# Autodesk Inventor assembly: ThermaShield
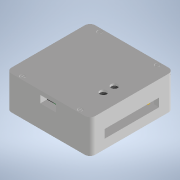
[picture p0: Inventor's stored thumbnail of the model, 180x180]
Saved by Autodesk Inventor 2022 (Build 260153000, 153)
## iProperties
Created: 2024-06-23
Part Number: ThermaShield
Document SubType Name: Assembly
Designer: Timur
Author: Timur
## Documents named in this file (8)
- B:\YandexDisk\YandexDisk\Учеба\НИУ ВШЭ\2 модуль\Проектный семинар\Финальный проект\Case\ThermaShield.iam
- B:\YandexDisk\YandexDisk\Учеба\НИУ ВШЭ\2 модуль\Проектный семинар\Финальный проект\Case\Case_Base.ipt
- B:\YandexDisk\YandexDisk\Учеба\НИУ ВШЭ\2 модуль\Проектный семинар\Финальный проект\Case\Threaded Insert - M2x4x3.5_Inventor.ipt
- B:\YandexDisk\YandexDisk\Учеба\НИУ ВШЭ\2 модуль\Проектный семинар\Финальный проект\Case\Стойка (M2x4)x5mm.ipt
- B:\YandexDisk\YandexDisk\Учеба\НИУ ВШЭ\2 модуль\Проектный семинар\Финальный проект\Case\Case_Cover.ipt
- B:\YandexDisk\YandexDisk\Учеба\НИУ ВШЭ\2 модуль\Проектный семинар\Финальный проект\Case\Винт M2-6gx6 ГОСТ 17475-80.ipt
- B:\YandexDisk\YandexDisk\Учеба\НИУ ВШЭ\2 модуль\Проектный семинар\Финальный проект\Case\Винт M2-6gx5 ГОСТ 1491-80.ipt
- B:\YandexDisk\YandexDisk\Учеба\НИУ ВШЭ\2 модуль\Проектный семинар\Финальный проект\Case\ThermaShield_V0.9\ThermaShield_V0.9.iam
## Components (23 placed, 7 different names)
1. Case_Base:1 — Совмещение:1, Заподлицо:1, Совмещение:2, Заподлицо:2, Совмещение:3, Заподлицо:3, Совмещение:4, Заподлицо:4, Совмещение:5, Совмещение:6, Совмещение:7, Совмещение:8, Заподлицо:5, Заподлицо:6, Заподлицо:7, Заподлицо:8, Заподлицо:9, Совмещение:20
2. Threaded Insert - M2x4x3.5_Inventor:1 — Совмещение:7, Заподлицо:7, Совмещение:12, Совмещение:13
3. Threaded Insert - M2x4x3.5_Inventor:2 — Совмещение:3, Заподлицо:3, Совмещение:22
4. Threaded Insert - M2x4x3.5_Inventor:3 — Совмещение:4, Заподлицо:4
5. Threaded Insert - M2x4x3.5_Inventor:4 — Совмещение:6, Заподлицо:6, Совмещение:11, Совмещение:14
6. Threaded Insert - M2x4x3.5_Inventor:5 — Совмещение:8, Заподлицо:8, Совмещение:10, Совмещение:15
7. Threaded Insert - M2x4x3.5_Inventor:6 — Совмещение:2, Заподлицо:2
8. Threaded Insert - M2x4x3.5_Inventor:7 — Совмещение:1, Заподлицо:1, Заподлицо:9, Совмещение:21
9. Threaded Insert - M2x4x3.5_Inventor:8 — Совмещение:5, Заподлицо:5, Совмещение:9, Совмещение:16
10. Стойка (M2x4)x5mm:1 — Совмещение:10, Совмещение:15
11. Стойка (M2x4)x5mm:2 — Совмещение:12, Совмещение:13, Совмещение:23, Совмещение:25
12. Стойка (M2x4)x5mm:3 — Совмещение:11, Совмещение:14
13. Стойка (M2x4)x5mm:4 — Совмещение:9, Совмещение:16
14. Case_Cover:1 — Совмещение:20, Совмещение:21, Совмещение:22, С поворотом:1, С поворотом:2, С поворотом:3, С поворотом:4
15. Винт ГОСТ 17475-80 M2 x 6:1 — С поворотом:4
16. Винт ГОСТ 17475-80 M2 x 6:2 — С поворотом:3
17. Винт ГОСТ 17475-80 M2 x 6:3 — С поворотом:2
18. Винт ГОСТ 17475-80 M2 x 6:4 — С поворотом:1
19. ThermaShield_V0.9:1 [sub-assembly] — Совмещение:23, Совмещение:25, Жесткий:1, Жесткий:2, С поворотом:5, Жесткий:3
20. Винт ГОСТ 1491-80 M 2 x 5:1 — С поворотом:5
21. Винт ГОСТ 1491-80 M 2 x 5:2 — Жесткий:1
22. Винт ГОСТ 1491-80 M 2 x 5:3 — Жесткий:3
23. Винт ГОСТ 1491-80 M 2 x 5:4 — Жесткий:2
## Relationships (38: Mate 21, Flush 9, RevoluteJoint 5, WeldJoint 3)
- Совмещение:1 [Mate]: Case_Base:1 ↔ Threaded Insert - M2x4x3.5_Inventor:7
- Заподлицо:1 [Flush]: Case_Base:1 ↔ Threaded Insert - M2x4x3.5_Inventor:7
- Совмещение:2 [Mate]: Case_Base:1 ↔ Threaded Insert - M2x4x3.5_Inventor:6
- Заподлицо:2 [Flush]: Case_Base:1 ↔ Threaded Insert - M2x4x3.5_Inventor:6
- Совмещение:3 [Mate]: Case_Base:1 ↔ Threaded Insert - M2x4x3.5_Inventor:2
- Заподлицо:3 [Flush]: Case_Base:1 ↔ Threaded Insert - M2x4x3.5_Inventor:2
- Совмещение:4 [Mate]: Case_Base:1 ↔ Threaded Insert - M2x4x3.5_Inventor:3
- Заподлицо:4 [Flush]: Case_Base:1 ↔ Threaded Insert - M2x4x3.5_Inventor:3
- Совмещение:5 [Mate]: Case_Base:1 ↔ Threaded Insert - M2x4x3.5_Inventor:8
- Совмещение:6 [Mate]: Case_Base:1 ↔ Threaded Insert - M2x4x3.5_Inventor:4
- Совмещение:7 [Mate]: Case_Base:1 ↔ Threaded Insert - M2x4x3.5_Inventor:1
- Совмещение:8 [Mate]: Case_Base:1 ↔ Threaded Insert - M2x4x3.5_Inventor:5
- Заподлицо:5 [Flush]: Case_Base:1 ↔ Threaded Insert - M2x4x3.5_Inventor:8
- Заподлицо:6 [Flush]: Case_Base:1 ↔ Threaded Insert - M2x4x3.5_Inventor:4
- Заподлицо:7 [Flush]: Case_Base:1 ↔ Threaded Insert - M2x4x3.5_Inventor:1
- Заподлицо:8 [Flush]: Case_Base:1 ↔ Threaded Insert - M2x4x3.5_Inventor:5
- Совмещение:9 [Mate]: Threaded Insert - M2x4x3.5_Inventor:8 ↔ Стойка (M2x4)x5mm:4
- Совмещение:10 [Mate]: Threaded Insert - M2x4x3.5_Inventor:5 ↔ Стойка (M2x4)x5mm:1
- Совмещение:11 [Mate]: Threaded Insert - M2x4x3.5_Inventor:4 ↔ Стойка (M2x4)x5mm:3
- Совмещение:12 [Mate]: Threaded Insert - M2x4x3.5_Inventor:1 ↔ Стойка (M2x4)x5mm:2
- Совмещение:13 [Mate]: Threaded Insert - M2x4x3.5_Inventor:1 ↔ Стойка (M2x4)x5mm:2
- Совмещение:14 [Mate]: Threaded Insert - M2x4x3.5_Inventor:4 ↔ Стойка (M2x4)x5mm:3
- Совмещение:15 [Mate]: Threaded Insert - M2x4x3.5_Inventor:5 ↔ Стойка (M2x4)x5mm:1
- Совмещение:16 [Mate]: Threaded Insert - M2x4x3.5_Inventor:8 ↔ Стойка (M2x4)x5mm:4
- Заподлицо:9 [Flush]: Case_Base:1 ↔ Threaded Insert - M2x4x3.5_Inventor:7
- Совмещение:20 [Mate]: Case_Base:1 ↔ Case_Cover:1
- Совмещение:21 [Mate]: Threaded Insert - M2x4x3.5_Inventor:7 ↔ Case_Cover:1
- Совмещение:22 [Mate]: Threaded Insert - M2x4x3.5_Inventor:2 ↔ Case_Cover:1
- С поворотом:1 [RevoluteJoint] (-6 mm): Case_Cover:1 ↔ Винт ГОСТ 17475-80 M2 x 6:4
- С поворотом:2 [RevoluteJoint] (-6 mm): Case_Cover:1 ↔ Винт ГОСТ 17475-80 M2 x 6:3
- С поворотом:3 [RevoluteJoint] (-6 mm): Case_Cover:1 ↔ Винт ГОСТ 17475-80 M2 x 6:2
- С поворотом:4 [RevoluteJoint] (-6 mm): Case_Cover:1 ↔ Винт ГОСТ 17475-80 M2 x 6:1
- Совмещение:23 [Mate]: Стойка (M2x4)x5mm:2 ↔ ThermaShield_V0.9:1
- Совмещение:25 [Mate]: Стойка (M2x4)x5mm:2 ↔ ThermaShield_V0.9:1
- Жесткий:1 [WeldJoint] (-5 mm): ThermaShield_V0.9:1 ↔ Винт ГОСТ 1491-80 M 2 x 5:2
- Жесткий:2 [WeldJoint] (-5 mm): ThermaShield_V0.9:1 ↔ Винт ГОСТ 1491-80 M 2 x 5:4
- С поворотом:5 [RevoluteJoint] (-5 mm): ThermaShield_V0.9:1 ↔ Винт ГОСТ 1491-80 M 2 x 5:1
- Жесткий:3 [WeldJoint] (-5 mm): ThermaShield_V0.9:1 ↔ Винт ГОСТ 1491-80 M 2 x 5:3
